# Autodesk Inventor assembly: DetectionRegionRender2
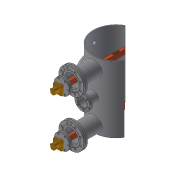
[picture p0: Inventor's stored thumbnail of the model, 180x180]
Saved by Autodesk Inventor 2015 SP1 (Build 190203100, 203)
## iProperties
Created: 2014-07-04
Part Number: DetectionRegionRender2
Document SubType Name: Assembly
Designer: I Rabey
Author: I Rabey
## Documents named in this file (10)
- C:\ColdMatter\CADFiles\EDM Machine\Detection Region\DetectionRegionRender2.iam
- C:\ColdMatter\CADFiles\EDM Machine\Detection Region\Detection Region Vacuum Collar.ipt
- C:\ColdMatter\CADFiles\EDM Machine\Detection Region\DN35CF Counter Bored.ipt
- C:\ColdMatter\CADFiles\EDM Machine\Detection Region\DN63CF Counter Bored.ipt
- C:\ColdMatter\CADFiles\EDM Machine\Detection Region\DN63CF Fixed Tapped Flange.ipt
- C:\ColdMatter\CADFiles\EDM Machine\Detection Region\DN16CF Fixed Tapped Flange.ipt
- C:\ColdMatter\CADFiles\EDM Machine\Detection Region\ISO200SS Bored K Flange.ipt
- C:\ColdMatter\CADFiles\EDM Machine\Detection Region\Microwave Transmission line\Microwave Waveguide Assembly\Microwave Waveguide Assembly.iam
- Microwave Waveguide Assembly.iam
- C:\ColdMatter\CADFiles\EDM Machine\Detection Region\molecularBeam.ipt
## Components (22 placed, 8 different names)
1. Detection Region Vacuum Collar:1 — Rotational:1, Rotational:3, Rotational:4, Rotational:5, Rotational:6, Rotational:7, Rotational:8, Rotational:9, Rotational:10, Rigid:2, Rotational:11, Rotational:12, Rotational:13, Rotational:14, Rotational:15, Rotational:16, Rotational:17, Rigid:3, Mate:2, Mate:3, Mate:4, Mate:6, Mate:7, Mate:9, Mate:10, Mate:11
2. DN35CF Counter Bored:1 — Rotational:1
3. DN63CF Counter Bored:1 — Rotational:17
4. DN35CF Counter Bored:2 — Rotational:3
5. DN63CF Counter Bored:2 — Rigid:3
6. DN63CF Fixed Tapped Flange:1 — Rotational:4
7. DN16CF Fixed Tapped Flange:1 — Rotational:5
8. DN63CF Fixed Tapped Flange:2 — Rotational:6
9. DN16CF Fixed Tapped Flange:2 — Rotational:7
10. DN35CF Counter Bored:3 — Rotational:8
11. DN63CF Counter Bored:3 — Rotational:9
12. DN35CF Counter Bored:4 — Rotational:10
13. DN63CF Counter Bored:4 — Rigid:2
14. DN63CF Fixed Tapped Flange:3 — Rotational:11
15. DN16CF Fixed Tapped Flange:3 — Rotational:12
16. DN63CF Fixed Tapped Flange:4 — Rotational:13
17. DN16CF Fixed Tapped Flange:4 — Rotational:14
18. ISO200SS Bored K Flange:1 — Rotational:15
19. ISO200SS Bored K Flange:2 — Rotational:16
20. Microwave Waveguide Assembly:1 [sub-assembly] — Mate:1, Mate:2, Flush:3, Flush:4
21. Microwave Waveguide Assembly:2 [sub-assembly] — Mate:5, Mate:6, Flush:2, Mate:8
22. molecularBeam:2 — Mate:15, Mate:16, Mate:17, Flush:5, Mate:18, Mate:19
## Relationships (44: Mate 19, RevoluteJoint 16, Flush 5, WeldJoint 2, Angle 2)
- Rotational:1 [RevoluteJoint]: Detection Region Vacuum Collar:1 ↔ DN35CF Counter Bored:1
- Rotational:3 [RevoluteJoint]: Detection Region Vacuum Collar:1 ↔ DN35CF Counter Bored:2
- Rotational:4 [RevoluteJoint]: Detection Region Vacuum Collar:1 ↔ DN63CF Fixed Tapped Flange:1
- Rotational:5 [RevoluteJoint]: Detection Region Vacuum Collar:1 ↔ DN16CF Fixed Tapped Flange:1
- Rotational:6 [RevoluteJoint]: Detection Region Vacuum Collar:1 ↔ DN63CF Fixed Tapped Flange:2
- Rotational:7 [RevoluteJoint]: Detection Region Vacuum Collar:1 ↔ DN16CF Fixed Tapped Flange:2
- Rotational:8 [RevoluteJoint]: Detection Region Vacuum Collar:1 ↔ DN35CF Counter Bored:3
- Rotational:9 [RevoluteJoint]: Detection Region Vacuum Collar:1 ↔ DN63CF Counter Bored:3
- Rotational:10 [RevoluteJoint]: Detection Region Vacuum Collar:1 ↔ DN35CF Counter Bored:4
- Rigid:2 [WeldJoint]: Detection Region Vacuum Collar:1 ↔ DN63CF Counter Bored:4
- Rotational:11 [RevoluteJoint]: Detection Region Vacuum Collar:1 ↔ DN63CF Fixed Tapped Flange:3
- Rotational:12 [RevoluteJoint]: Detection Region Vacuum Collar:1 ↔ DN16CF Fixed Tapped Flange:3
- Rotational:13 [RevoluteJoint]: Detection Region Vacuum Collar:1 ↔ DN63CF Fixed Tapped Flange:4
- Rotational:14 [RevoluteJoint]: Detection Region Vacuum Collar:1 ↔ DN16CF Fixed Tapped Flange:4
- Rotational:15 [RevoluteJoint]: Detection Region Vacuum Collar:1 ↔ ISO200SS Bored K Flange:1
- Rotational:16 [RevoluteJoint]: Detection Region Vacuum Collar:1 ↔ ISO200SS Bored K Flange:2
- Rotational:17 [RevoluteJoint]: Detection Region Vacuum Collar:1 ↔ DN63CF Counter Bored:1
- Rigid:3 [WeldJoint]: Detection Region Vacuum Collar:1 ↔ DN63CF Counter Bored:2
- Mate:1: Microwave Waveguide Assembly:1
- Mate:2: Detection Region Vacuum Collar:1 ↔ Microwave Waveguide Assembly:1
- Mate:3: Detection Region Vacuum Collar:1
- Mate:4: Detection Region Vacuum Collar:1
- Mate:5: Microwave Waveguide Assembly:2
- Mate:6: Detection Region Vacuum Collar:1 ↔ Microwave Waveguide Assembly:2
- Flush:2 (-71 mm): Microwave Waveguide Assembly:2
- Mate:7: Detection Region Vacuum Collar:1
- Mate:8: Microwave Waveguide Assembly:2
- Angle:1 (135 deg)
- Flush:3 (-71 mm): Microwave Waveguide Assembly:1
- Mate:9: Detection Region Vacuum Collar:1
- Flush:4 (-170 mm): Microwave Waveguide Assembly:1
- Mate:10: Detection Region Vacuum Collar:1
- Mate:11: Detection Region Vacuum Collar:1
- Mate:12
- Mate:13
- Mate:14
- Angle:2 (0 deg)
- Mate:15: molecularBeam:2
- Mate:16: molecularBeam:2
- Mate:17: molecularBeam:2
- Flush:5: molecularBeam:2
- Mate:18: molecularBeam:2
- Flush:6 (-480 mm)
- Mate:19: molecularBeam:2
